# Autodesk Inventor assembly: EncoderAssembly
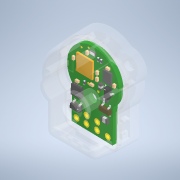
[picture p0: Inventor's stored thumbnail of the model, 180x180]
Saved by Autodesk Inventor 2020 (Build 240168000, 168)
## iProperties
Created: 2021-02-20
Part Number: EncoderAssembly
Document SubType Name: Assembly
Designer: turnm
Author: turnm
## Documents named in this file (3)
- C:\Users\turnm\Documents\GrabCAD\Infinite Recharge 2020\Build season\EncoderCAD\EncoderAssembly.iam
- C:\Users\turnm\Downloads\Cancoder_CAD\Housing.ipt
- C:\Users\turnm\Downloads\Cancoder_CAD\PCB Assembly.ipt
## Components (2 placed, 2 different names)
1. Housing:1 — Mate:1, Flush:1
2. PCB Assembly:1 — Mate:1, Flush:1
## Relationships (2: Mate 1, Flush 1)
- Mate:1: Housing:1 ↔ PCB Assembly:1
- Flush:1 (7.112 mm): Housing:1 ↔ PCB Assembly:1
